# Autodesk Inventor assembly: front wheels
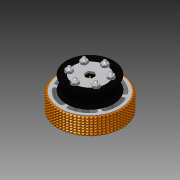
[picture p0: Inventor's stored thumbnail of the model, 180x180]
Saved by Autodesk Inventor 2014 SP1 (Build 180222100, 222)
## iProperties
Created: 2014-01-05
Part Number: front wheels
Document SubType Name: Assembly
Designer: Arpan
Mass: 337.424 g
Surface Area: 996.082 cm^2
Volume: 144.882 cm^3
Density: 2.32897 g/cm^3
Author: Arpan
## Documents named in this file (7)
- C:\Users\Arpan\Documents\GitHub\2014buildCAD\chassisdrivetrain\chassis light\COTS items\front wheels.iam
- C:\Users\Arpan\Documents\GitHub\2014buildCAD\chassisdrivetrain\chassis light\COTS items\4 Perf ThruTread 500 Hex (1).ipt
- C:\Users\Arpan\Documents\GitHub\2014buildCAD\chassisdrivetrain\chassis light\COTS items\4 Inch Performance Wheel Tread.ipt
- C:\Users\Arpan\Documents\GitHub\2014buildCAD\chassisdrivetrain\chassis light\COTS items\DBK_42ToothPulley V2.iam
- C:\Users\Arpan\Documents\GitHub\2014buildCAD\hardware\10-24\2 inch screw 90044A116.ipt
- C:\Users\Arpan\Documents\GitHub\2014buildCAD\hardware\10-24\thin hex locknut 90633A011.ipt
- C:\Users\Arpan\Documents\GitHub\2014buildCAD\chassisdrivetrain\chassis light\chassis hex hub clone.ipt
## Components (16 placed, 6 different names)
1. 4 Perf ThruTread 500 Hex (1):1 — Mate:1, Mate:2, Mate:19, Mate:20, Mate:21, Mate:22, Mate:23, Mate:24, Mate:25, Mate:26, Mate:27, Mate:28, Mate:29, Mate:30
2. 4 Inch Performance Wheel Tread:1 — Mate:1, Mate:2
3. DBK_42ToothPulley V2:1 [sub-assembly] — Mate:43, Mate:44, Mate:45
4. 2 inch screw 90044A116:1 — Mate:21, Mate:22, Mate:34
5. 2 inch screw 90044A116:2 — Mate:19, Mate:20, Mate:36
6. 2 inch screw 90044A116:3 — Mate:27, Mate:28, Mate:40
7. 2 inch screw 90044A116:4 — Mate:23, Mate:24, Mate:32
8. 2 inch screw 90044A116:5 — Mate:25, Mate:26, Mate:42
9. 2 inch screw 90044A116:6 — Mate:29, Mate:30, Mate:38
10. thin hex locknut 90633A011:1 — Mate:34, Mate:47
11. thin hex locknut 90633A011:2 — Mate:42, Mate:51
12. thin hex locknut 90633A011:3 — Mate:32, Mate:48
13. thin hex locknut 90633A011:4 — Mate:36, Mate:46
14. thin hex locknut 90633A011:5 — Mate:40, Mate:50
15. thin hex locknut 90633A011:6 — Mate:38, Mate:49
16. chassis hex hub clone:1 — Mate:43, Mate:44, Mate:45, Mate:46, Mate:47, Mate:48, Mate:49, Mate:50, Mate:51
## Relationships (29: Mate 29)
- Mate:1: 4 Perf ThruTread 500 Hex (1):1 ↔ 4 Inch Performance Wheel Tread:1
- Mate:2: 4 Perf ThruTread 500 Hex (1):1 ↔ 4 Inch Performance Wheel Tread:1
- Mate:19: 4 Perf ThruTread 500 Hex (1):1 ↔ 2 inch screw 90044A116:2
- Mate:20: 4 Perf ThruTread 500 Hex (1):1 ↔ 2 inch screw 90044A116:2
- Mate:21: 4 Perf ThruTread 500 Hex (1):1 ↔ 2 inch screw 90044A116:1
- Mate:22: 4 Perf ThruTread 500 Hex (1):1 ↔ 2 inch screw 90044A116:1
- Mate:23: 4 Perf ThruTread 500 Hex (1):1 ↔ 2 inch screw 90044A116:4
- Mate:24: 4 Perf ThruTread 500 Hex (1):1 ↔ 2 inch screw 90044A116:4
- Mate:25: 4 Perf ThruTread 500 Hex (1):1 ↔ 2 inch screw 90044A116:5
- Mate:26: 4 Perf ThruTread 500 Hex (1):1 ↔ 2 inch screw 90044A116:5
- Mate:27: 4 Perf ThruTread 500 Hex (1):1 ↔ 2 inch screw 90044A116:3
- Mate:28: 4 Perf ThruTread 500 Hex (1):1 ↔ 2 inch screw 90044A116:3
- Mate:29: 4 Perf ThruTread 500 Hex (1):1 ↔ 2 inch screw 90044A116:6
- Mate:30: 4 Perf ThruTread 500 Hex (1):1 ↔ 2 inch screw 90044A116:6
- Mate:32: 2 inch screw 90044A116:4 ↔ thin hex locknut 90633A011:3
- Mate:34: 2 inch screw 90044A116:1 ↔ thin hex locknut 90633A011:1
- Mate:36: 2 inch screw 90044A116:2 ↔ thin hex locknut 90633A011:4
- Mate:38: 2 inch screw 90044A116:6 ↔ thin hex locknut 90633A011:6
- Mate:40: 2 inch screw 90044A116:3 ↔ thin hex locknut 90633A011:5
- Mate:42: 2 inch screw 90044A116:5 ↔ thin hex locknut 90633A011:2
- Mate:43: DBK_42ToothPulley V2:1 ↔ chassis hex hub clone:1
- Mate:44: DBK_42ToothPulley V2:1 ↔ chassis hex hub clone:1
- Mate:45: DBK_42ToothPulley V2:1 ↔ chassis hex hub clone:1
- Mate:46: thin hex locknut 90633A011:4 ↔ chassis hex hub clone:1
- Mate:47: thin hex locknut 90633A011:1 ↔ chassis hex hub clone:1
- Mate:48: thin hex locknut 90633A011:3 ↔ chassis hex hub clone:1
- Mate:49: thin hex locknut 90633A011:6 ↔ chassis hex hub clone:1
- Mate:50: thin hex locknut 90633A011:5 ↔ chassis hex hub clone:1
- Mate:51: thin hex locknut 90633A011:2 ↔ chassis hex hub clone:1
